# Autodesk Inventor assembly: LeftTractionWheelsDTA
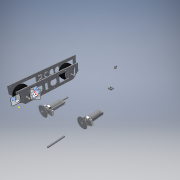
[picture p0: Inventor's stored thumbnail of the model, 180x180]
Saved by Autodesk Inventor 2017 (Build 210142000, 142)
## iProperties
Created: 2017-08-16
Part Number: LeftTractionWheelsDTA
Document SubType Name: Assembly
Designer: User
Author: User
## Documents named in this file (11)
- C:\Robotics\CAD\2016-17_CAD\Sub-Assemblies\LeftTractionWheelsDTA.iam
- C:\Robotics\CAD\2016-17_CAD\DriveTrain\drive train standoff.ipt
- C:\Robotics\CAD\2016-17_CAD\DriveTrain\DrainTrainPlate2.0LeftOutside.iam
- C:\Robotics\CAD\2016-17_CAD\DriveTrain\DriveTrainPlate2.0LeftInside.ipt
- C:\Robotics\CAD\COTSParts\Motors\Andymark 2964  NeveRest 40 Motor.ipt
- C:\Robotics\CAD\COTSParts\Tetrix\tetrix-motor-mounts-1.snapshot.1\Tetrex 2pc motor mount.ipt
- C:\Robotics\CAD\COTSParts\Actobotics\615 parts\615114.ipt
- C:\Robotics\CAD\COTSParts\Actobotics\545 parts\545456.ipt
- C:\Robotics\CAD\COTSParts\Actobotics\545 parts\545556.ipt
- C:\Robotics\CAD\COTSParts\Actobotics\634 parts\634080.ipt
- C:\Robotics\CAD\COTSParts\Wheels\4in Wheel Intergreated Hub 8mm Rev2.ipt
## Components (29 placed, 10 different names)
1. drive train standoff:1
2. drive train standoff:2
3. drive train standoff:3
4. DrainTrainPlate2.0LeftOutside:1 [sub-assembly] — Mate:30, Flush:1, Mate:31, Flush:2, Flush:3
5. DriveTrainPlate2.0LeftInside:1 — Mate:28, Mate:29, Flush:1, Mate:32, Mate:33
6. Andymark 2964  NeveRest 40 Motor:1 — Mate:35, Mate:39, Mate:41
7. Andymark 2964  NeveRest 40 Motor:2 — Mate:34, Mate:36
8. Tetrex 2pc motor mount:1 — Mate:35
9. Tetrex 2pc motor mount:2 — Mate:34
10. 615114:1 — Mate:6, Mate:7, Mate:29
11. 615114:2 — Mate:40, Mate:41
12. 615114:3 — Mate:17, Mate:18, Mate:32
13. 615114:4 — Mate:37, Flush:4
14. 545456:1 — Mate:19, Mate:20, Mate:21
15. 545456:2 — Mate:13, Mate:14, Mate:15
16. 545456:3 — Mate:2, Mate:3, Mate:4
17. 545456:4 — Mate:8, Mate:9, Mate:10, Mate:25
18. 545556:1 — Mate:15, Mate:16, Mate:17
19. 545556:2 — Mate:4, Mate:5, Mate:6
20. 545556:3 — Mate:39, Mate:40
21. 545556:4 — Mate:36, Mate:37, Flush:4
22. 634080:1 — Mate:12, Mate:14, Mate:16, Mate:18, Mate:20, Mate:22, Mate:33, Flush:3
23. 634080:2 — Mate:1, Mate:3, Mate:5, Mate:7, Mate:9, Mate:26, Mate:28, Mate:31, Flush:2
24. 545556:5
25. 545556:6 — Mate:21, Mate:22
26. 4in Wheel Intergreated Hub 8mm Rev2:1 — Mate:1, Mate:2, Mate:8
27. 4in Wheel Intergreated Hub 8mm Rev2:2 — Mate:12, Mate:13, Mate:19
28. 545556:7 — Mate:25, Mate:26, Mate:30
29. 545556:8 — Mate:10
## Relationships (40: Mate 36, Flush 4)
- Mate:1: 634080:2 ↔ 4in Wheel Intergreated Hub 8mm Rev2:1
- Mate:2: 545456:3 ↔ 4in Wheel Intergreated Hub 8mm Rev2:1
- Mate:3: 545456:3 ↔ 634080:2
- Mate:4: 545456:3 ↔ 545556:2
- Mate:5: 545556:2 ↔ 634080:2
- Mate:6: 615114:1 ↔ 545556:2
- Mate:7: 615114:1 ↔ 634080:2
- Mate:8: 545456:4 ↔ 4in Wheel Intergreated Hub 8mm Rev2:1
- Mate:9: 545456:4 ↔ 634080:2
- Mate:10: 545456:4 ↔ 545556:8
- Mate:12: 634080:1 ↔ 4in Wheel Intergreated Hub 8mm Rev2:2
- Mate:13: 545456:2 ↔ 4in Wheel Intergreated Hub 8mm Rev2:2
- Mate:14: 545456:2 ↔ 634080:1
- Mate:15: 545456:2 ↔ 545556:1
- Mate:16: 545556:1 ↔ 634080:1
- Mate:17: 615114:3 ↔ 545556:1
- Mate:18: 615114:3 ↔ 634080:1
- Mate:19: 545456:1 ↔ 4in Wheel Intergreated Hub 8mm Rev2:2
- Mate:20: 545456:1 ↔ 634080:1
- Mate:21: 545456:1 ↔ 545556:6
- Mate:22: 634080:1 ↔ 545556:6
- Mate:25: 545456:4 ↔ 545556:7
- Mate:26: 634080:2 ↔ 545556:7
- Mate:28: DriveTrainPlate2.0LeftInside:1 ↔ 634080:2
- Mate:29 (6.35 mm): DriveTrainPlate2.0LeftInside:1 ↔ 615114:1
- Mate:30 (6.35 mm): DrainTrainPlate2.0LeftOutside:1 ↔ 545556:7
- Flush:1: DrainTrainPlate2.0LeftOutside:1 ↔ DriveTrainPlate2.0LeftInside:1
- Mate:31: DrainTrainPlate2.0LeftOutside:1 ↔ 634080:2
- Flush:2: DrainTrainPlate2.0LeftOutside:1 ↔ 634080:2
- Mate:32 (6.35 mm): DriveTrainPlate2.0LeftInside:1 ↔ 615114:3
- Mate:33: DriveTrainPlate2.0LeftInside:1 ↔ 634080:1
- Flush:3: DrainTrainPlate2.0LeftOutside:1 ↔ 634080:1
- Mate:34: Andymark 2964  NeveRest 40 Motor:2 ↔ Tetrex 2pc motor mount:2
- Mate:35: Andymark 2964  NeveRest 40 Motor:1 ↔ Tetrex 2pc motor mount:1
- Mate:36: Andymark 2964  NeveRest 40 Motor:2 ↔ 545556:4
- Mate:37: 615114:4 ↔ 545556:4
- Flush:4: 615114:4 ↔ 545556:4
- Mate:39: Andymark 2964  NeveRest 40 Motor:1 ↔ 545556:3
- Mate:40: 615114:2 ↔ 545556:3
- Mate:41: Andymark 2964  NeveRest 40 Motor:1 ↔ 615114:2
